# Autodesk Inventor assembly: 1_Base
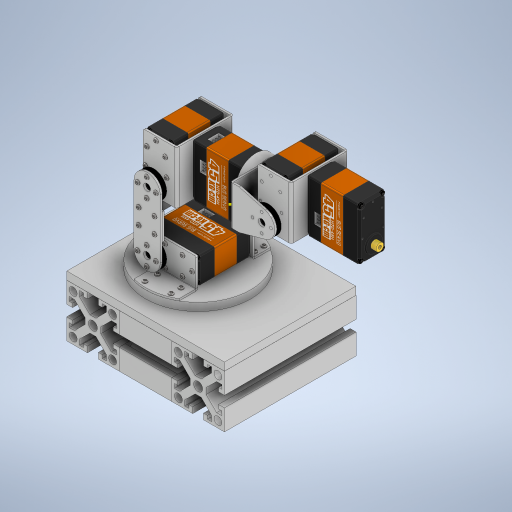
[picture p0: Inventor's stored thumbnail of the model, 512x512]
Saved by Autodesk Inventor 2024.1 (Build 281209000, 209)
## iProperties
Created: 2023-08-24
Part Number: 1_Base
Document SubType Name: Assembly
Designer: chanh
Author: chanh
## Documents named in this file (28)
- C:\Users\chanh\OneDrive - 연세대학교 (Yonsei University)\로봇\Humanoid\Roboin Humanoid Project\Inventor\rh_plus_7_axis_robot_arm_hardware\Assembly\2_Arm.iam
- C:\Users\chanh\OneDrive - 연세대학교 (Yonsei University)\로봇\Humanoid\Roboin Humanoid Project\Inventor\rh_plus_7_axis_robot_arm_hardware\Part\HTD-45H, Horn\HTD-45H\HTD-45H.ipt
- C:\Users\chanh\OneDrive - 연세대학교 (Yonsei University)\로봇\Humanoid\Roboin Humanoid Project\Inventor\rh_plus_7_axis_robot_arm_hardware\Part\Frame\axis_1_top_frame.ipt
- C:\Users\chanh\OneDrive - 연세대학교 (Yonsei University)\로봇\Humanoid\Roboin Humanoid Project\Inventor\rh_plus_7_axis_robot_arm_hardware\Part\Other Parts\Aluminum_Profile_4040_100.14mm_top.ipt
- C:\Users\chanh\OneDrive - 연세대학교 (Yonsei University)\로봇\Humanoid\Roboin Humanoid Project\Inventor\rh_plus_7_axis_robot_arm_hardware\Part\Other Parts\Aluminum_Profile_4040_40.10mm_right.ipt
- C:\Users\chanh\OneDrive - 연세대학교 (Yonsei University)\로봇\Humanoid\Roboin Humanoid Project\Inventor\rh_plus_7_axis_robot_arm_hardware\Part\Other Parts\Aluminum_Profile_4040_40.10mm_left.ipt
- C:\Users\chanh\OneDrive - 연세대학교 (Yonsei University)\로봇\Humanoid\Roboin Humanoid Project\Inventor\rh_plus_7_axis_robot_arm_hardware\Part\Other Parts\Aluminum_Profile_4040_100.14mm_bottom.ipt
- C:\Users\chanh\OneDrive - 연세대학교 (Yonsei University)\로봇\Humanoid\Roboin Humanoid Project\Inventor\rh_plus_7_axis_robot_arm_hardware\Part\HTD-45H, Horn\HTD-45H\M2x32.ipt
- C:\Users\chanh\OneDrive - 연세대학교 (Yonsei University)\로봇\Humanoid\Roboin Humanoid Project\Inventor\rh_plus_7_axis_robot_arm_hardware\Part\HTD-45H, Horn\Horn\Top Horn.ipt
- C:\Users\chanh\OneDrive - 연세대학교 (Yonsei University)\로봇\Humanoid\Roboin Humanoid Project\Inventor\rh_plus_7_axis_robot_arm_hardware\Part\Bolt, Bearing\M2x6 Round Bolt.ipt
- C:\Users\chanh\OneDrive - 연세대학교 (Yonsei University)\로봇\Humanoid\Roboin Humanoid Project\Inventor\rh_plus_7_axis_robot_arm_hardware\Part\Bolt, Bearing\M2x35 Round Bolt.ipt
- C:\Users\chanh\OneDrive - 연세대학교 (Yonsei University)\로봇\Humanoid\Roboin Humanoid Project\Inventor\rh_plus_7_axis_robot_arm_hardware\Part\Frame\axis_2_bottom_frame.ipt
- C:\Users\chanh\OneDrive - 연세대학교 (Yonsei University)\로봇\Humanoid\Roboin Humanoid Project\Inventor\rh_plus_7_axis_robot_arm_hardware\Part\Bolt, Bearing\AXK5070+AS Bearing.ipt
- C:\Users\chanh\OneDrive - 연세대학교 (Yonsei University)\로봇\Humanoid\Roboin Humanoid Project\Inventor\rh_plus_7_axis_robot_arm_hardware\Part\Bolt, Bearing\M2x6 Bolt.ipt
- C:\Users\chanh\OneDrive - 연세대학교 (Yonsei University)\로봇\Humanoid\Roboin Humanoid Project\Inventor\rh_plus_7_axis_robot_arm_hardware\Part\HTD-45H, Horn\HTD-45H\HTD-45H.iam
- C:\Users\chanh\OneDrive - 연세대학교 (Yonsei University)\로봇\Humanoid\Roboin Humanoid Project\Inventor\rh_plus_7_axis_robot_arm_hardware\Part\HTD-45H, Horn\Horn\M3x6.ipt
- C:\Users\chanh\OneDrive - 연세대학교 (Yonsei University)\로봇\Humanoid\Roboin Humanoid Project\Inventor\rh_plus_7_axis_robot_arm_hardware\Part\Frame\axis_2_bottom_L_frame(top).ipt
- C:\Users\chanh\OneDrive - 연세대학교 (Yonsei University)\로봇\Humanoid\Roboin Humanoid Project\Inventor\rh_plus_7_axis_robot_arm_hardware\Part\Frame\axis_2_bottom_L_frame(bottom).ipt
- C:\Users\chanh\OneDrive - 연세대학교 (Yonsei University)\로봇\Humanoid\Roboin Humanoid Project\Inventor\rh_plus_7_axis_robot_arm_hardware\Part\HTD-45H, Horn\Horn\Bottom Horn.ipt
- C:\Users\chanh\OneDrive - 연세대학교 (Yonsei University)\로봇\Humanoid\Roboin Humanoid Project\Inventor\rh_plus_7_axis_robot_arm_hardware\Part\Bolt, Bearing\M2x4 Round Bolt.ipt
- C:\Users\chanh\OneDrive - 연세대학교 (Yonsei University)\로봇\Humanoid\Roboin Humanoid Project\Inventor\rh_plus_7_axis_robot_arm_hardware\Part\Frame\axis_3_bottom_frame(top).ipt
- C:\Users\chanh\OneDrive - 연세대학교 (Yonsei University)\로봇\Humanoid\Roboin Humanoid Project\Inventor\rh_plus_7_axis_robot_arm_hardware\Part\Frame\axis_3_bottom_frame(bottom).ipt
- C:\Users\chanh\OneDrive - 연세대학교 (Yonsei University)\로봇\Humanoid\Roboin Humanoid Project\Inventor\rh_plus_7_axis_robot_arm_hardware\Part\Frame\axis_3_bottom_frame(middle).ipt
- C:\Users\chanh\OneDrive - 연세대학교 (Yonsei University)\로봇\Humanoid\Roboin Humanoid Project\Inventor\rh_plus_7_axis_robot_arm_hardware\Part\Frame\axis_3_top_frame.ipt
- C:\Users\chanh\OneDrive - 연세대학교 (Yonsei University)\로봇\Humanoid\Roboin Humanoid Project\Inventor\rh_plus_7_axis_robot_arm_hardware\Part\Frame\axis_4_top_frame.ipt
- C:\Users\chanh\OneDrive - 연세대학교 (Yonsei University)\로봇\Humanoid\Roboin Humanoid Project\Inventor\rh_plus_7_axis_robot_arm_hardware\Part\Bolt, Bearing\2030 Teflon Sheet.ipt
- C:\Users\chanh\OneDrive - 연세대학교 (Yonsei University)\로봇\Humanoid\Roboin Humanoid Project\Inventor\rh_plus_7_axis_robot_arm_hardware\Part\Frame\axis_5_bottom_frame.ipt
- C:\Users\chanh\OneDrive - 연세대학교 (Yonsei University)\로봇\Humanoid\Roboin Humanoid Project\Inventor\rh_plus_7_axis_robot_arm_hardware\Part\Frame\axis_5_top_frame.ipt
## Components (113 placed, 26 different names)
1. Aluminum_Profile_4040_100.14mm_top:1 — Flush:13, Flush:14, Mate:2, Mate:3, Flush:15, Flush:16, Mate:4, Flush:17, Flush:18, Mate:6
2. Aluminum_Profile_4040_40.10mm_right:1 — Mate:3, Flush:15, Flush:16
3. Aluminum_Profile_4040_40.10mm_left:1 — Mate:4, Flush:17, Flush:18, Mate:5, Flush:20
4. Aluminum_Profile_4040_100.14mm_bottom:1 — Flush:19, Mate:5, Flush:20
5. HTD-45H:1 — Mate:1, Flush:1, Flush:2, Flush:12, Flush:13, Flush:14, Mate:2, Flush:19, Rigid:1, Rigid:2, Rotational:1, Mate:7, Mate:8
6. axis_1_top_frame:1 — Flush:11, Flush:12, Mate:6, Rigid:11, Rigid:12, Rigid:13, Rigid:14, Rigid:15, Rigid:16, Rigid:17, Mate:9
7. HTD-45H:2 [sub-assembly] — Flush:21, Mate:11, Flush:23, Flush:24, Mate:13, Mate:17, Rotational:2
8. axis_2_bottom_frame:1 — Rigid:10, Rigid:18, Rigid:19, Rigid:20, Rigid:21, Flush:21, Mate:11, Mate:14
9. axis_2_bottom_L_frame(top):1 — Flush:23, Flush:24, Mate:13, Mate:14, Rigid:23, Rigid:24, Rigid:25, Rigid:26, Rigid:27, Rigid:28, Rigid:29, Rigid:30, Rigid:31
10. axis_2_bottom_L_frame(bottom):1 — Mate:17, Rigid:32, Rigid:33, Rigid:34, Rigid:35, Rigid:36, Rigid:37, Rigid:38, Rigid:39, Rigid:40, Rigid:41, Rigid:42, Rigid:43
11. HTD-45H:3 [sub-assembly] — Rotational:3, Flush:25, Mate:18, Flush:26
12. axis_3_bottom_frame(top):1 — Rigid:44, Rigid:45, Rigid:48, Rigid:49, Rigid:50, Rigid:51, Rigid:52, Rigid:53, Rigid:54, Rigid:55, Rigid:56, Rigid:57, Rigid:58, Rigid:59, Rigid:60
13. axis_3_bottom_frame(middle):1 — Rigid:48, Rigid:104
14. axis_3_bottom_frame(bottom):1 — Rigid:61, Rigid:62, Rigid:63, Rigid:64, Rigid:65, Rigid:66, Rigid:67, Rigid:68, Rigid:69, Rigid:70, Rigid:71, Rigid:72, Rigid:102, Rigid:103, Rigid:104
15. axis_3_top_frame:1 — Flush:25, Mate:18, Flush:26, Rigid:74, Rigid:75, Rigid:76, Rigid:77, Rigid:78, Rigid:79, Rigid:80, Rigid:81, Rigid:82, Rigid:83, Rigid:84, Rigid:85, Rigid:86, Rigid:87, Rigid:88, Rigid:89, Rigid:90
16. HTD-45H:4 — Rigid:90, Rigid:91, Rigid:92, Angle:1, Mate:20, Rotational:4
17. 2030 Teflon Sheet:1 — Rigid:97
18. axis_4_top_frame:1 — Angle:1, Mate:20, Rigid:93, Rigid:94, Rigid:95, Rigid:96, Rigid:97
19. HTD-45H:5 [sub-assembly] — Rotational:5, Rigid:105
20. 2030 Teflon Sheet:2
21. axis_5_bottom_frame:1 — Rigid:99, Rigid:100, Rigid:101
22. axis_5_top_frame:1 — Rigid:105, Mate:21, Flush:27, Mate:22
23. HTD-45H:6 [sub-assembly] — Mate:21, Flush:27, Mate:22
24. M2x32:1 — Rigid:2
25. M2x32:2 — Rigid:1
26. Top Horn:1 — Rotational:1, Rigid:10, Rigid:22
27. M3x6:1 — Rigid:22
28. M2x6 Round Bolt:3 — Rigid:16
29. M2x6 Round Bolt:4 — Rigid:17
30. M2x6 Round Bolt:5 — Rigid:15
31. AXK5070+AS Bearing:1 — Mate:7, Mate:8, Mate:9
32. M2x6 Round Bolt:1 — Rigid:14
33. M2x6 Round Bolt:2 — Rigid:13
34. M2x35 Round Bolt:1 — Rigid:11
35. M2x35 Round Bolt:2 — Rigid:12
36. Bottom Horn:5 — Rigid:102
37. Top Horn:2 — Rotational:2, Rigid:44
38. M2x6 Bolt:1 — Rigid:18
39. M2x6 Bolt:2 — Rigid:19
40. M2x6 Bolt:3 — Rigid:20
41. M2x6 Bolt:4 — Rigid:21
42. M2x4 Round Bolt:1 — Rigid:23
43. M2x4 Round Bolt:2 — Rigid:24
44. M2x4 Round Bolt:3 — Rigid:25
45. M2x4 Round Bolt:4 — Rigid:26
46. M2x4 Round Bolt:5 — Rigid:27
47. M2x4 Round Bolt:6 — Rigid:28
48. M2x4 Round Bolt:7 — Rigid:29
49. M2x4 Round Bolt:8 — Rigid:30
50. M2x4 Round Bolt:9 — Rigid:31
51. M2x4 Round Bolt:10 — Rigid:32
52. M2x4 Round Bolt:11 — Rigid:33
53. M2x4 Round Bolt:12 — Rigid:34
54. M2x4 Round Bolt:13 — Rigid:35
55. M2x4 Round Bolt:14 — Rigid:36
56. M2x4 Round Bolt:15 — Rigid:37
57. M2x4 Round Bolt:16 — Rigid:38
58. M2x4 Round Bolt:17 — Rigid:39
59. M2x4 Round Bolt:18 — Rigid:40
60. M2x4 Round Bolt:19 — Rigid:41
61. M2x4 Round Bolt:20 — Rigid:42
62. M2x4 Round Bolt:21 — Rigid:43
63. Bottom Horn:4 — Rigid:103
64. Top Horn:3 — Rotational:3, Rigid:45
65. M2x4 Round Bolt:22 — Rigid:50
66. M2x4 Round Bolt:23 — Rigid:51
67. M2x4 Round Bolt:24 — Rigid:52
68. M2x4 Round Bolt:25 — Rigid:49
69. M2x4 Round Bolt:26 — Rigid:53
70. M2x4 Round Bolt:27 — Rigid:54
71. M2x4 Round Bolt:28 — Rigid:55
72. M2x4 Round Bolt:29 — Rigid:56
73. M2x4 Round Bolt:30 — Rigid:57
74. M2x4 Round Bolt:31 — Rigid:58
75. M2x4 Round Bolt:32 — Rigid:59
76. M2x4 Round Bolt:33 — Rigid:60
77. M2x4 Round Bolt:34 — Rigid:61
78. M2x4 Round Bolt:35 — Rigid:62
79. M2x4 Round Bolt:36 — Rigid:63
80. M2x4 Round Bolt:37 — Rigid:64
81. M2x4 Round Bolt:38 — Rigid:65
82. M2x4 Round Bolt:39 — Rigid:66
83. M2x4 Round Bolt:40 — Rigid:67
84. M2x4 Round Bolt:41 — Rigid:68
85. M2x4 Round Bolt:42 — Rigid:69
86. M2x4 Round Bolt:43 — Rigid:70
87. M2x4 Round Bolt:44 — Rigid:71
88. M2x4 Round Bolt:45 — Rigid:72
89. M2x4 Round Bolt:46 — Rigid:74
90. M2x4 Round Bolt:47 — Rigid:75
91. M2x4 Round Bolt:48 — Rigid:76
92. M2x4 Round Bolt:49 — Rigid:77
93. M2x4 Round Bolt:50 — Rigid:78
94. M2x4 Round Bolt:51 — Rigid:79
95. M2x4 Round Bolt:52 — Rigid:80
96. M2x4 Round Bolt:53 — Rigid:81
97. M2x4 Round Bolt:54 — Rigid:82
98. M2x4 Round Bolt:55 — Rigid:83
99. M2x4 Round Bolt:56 — Rigid:84
100. M2x4 Round Bolt:57 — Rigid:85
101. M2x4 Round Bolt:58 — Rigid:86
102. M2x4 Round Bolt:59 — Rigid:87
103. M2x4 Round Bolt:60 — Rigid:88
104. M2x4 Round Bolt:61 — Rigid:89
105. Top Horn:6 — Rotational:4, Rigid:99
106. M2x32:3 — Rigid:92
107. M2x32:4 — Rigid:91
108. M2x6 Round Bolt:6 — Rigid:93
109. M2x6 Round Bolt:7 — Rigid:94
110. M2x35 Round Bolt:3 — Rigid:95
111. M2x35 Round Bolt:4 — Rigid:96
112. Top Horn:7 — Rigid:100, Rotational:5
113. Bottom Horn:3 — Rigid:101
## Relationships (135: WeldJoint 94, Flush 18, Mate 17, RevoluteJoint 5, Angle 1)
- Mate:1: HTD-45H:1
- Flush:1: HTD-45H:1
- Flush:2: HTD-45H:1
- Flush:11: axis_1_top_frame:1
- Flush:12: HTD-45H:1 ↔ axis_1_top_frame:1
- Flush:13: Aluminum_Profile_4040_100.14mm_top:1 ↔ HTD-45H:1
- Flush:14: Aluminum_Profile_4040_100.14mm_top:1 ↔ HTD-45H:1
- Mate:2: Aluminum_Profile_4040_100.14mm_top:1 ↔ HTD-45H:1
- Mate:3: Aluminum_Profile_4040_100.14mm_top:1 ↔ Aluminum_Profile_4040_40.10mm_right:1
- Flush:15: Aluminum_Profile_4040_100.14mm_top:1 ↔ Aluminum_Profile_4040_40.10mm_right:1
- Flush:16: Aluminum_Profile_4040_100.14mm_top:1 ↔ Aluminum_Profile_4040_40.10mm_right:1
- Mate:4: Aluminum_Profile_4040_100.14mm_top:1 ↔ Aluminum_Profile_4040_40.10mm_left:1
- Flush:17: Aluminum_Profile_4040_100.14mm_top:1 ↔ Aluminum_Profile_4040_40.10mm_left:1
- Flush:18: Aluminum_Profile_4040_100.14mm_top:1 ↔ Aluminum_Profile_4040_40.10mm_left:1
- Flush:19: Aluminum_Profile_4040_100.14mm_bottom:1 ↔ HTD-45H:1
- Mate:5: Aluminum_Profile_4040_40.10mm_left:1 ↔ Aluminum_Profile_4040_100.14mm_bottom:1
- Flush:20: Aluminum_Profile_4040_40.10mm_left:1 ↔ Aluminum_Profile_4040_100.14mm_bottom:1
- Mate:6: Aluminum_Profile_4040_100.14mm_top:1 ↔ axis_1_top_frame:1
- Rigid:1 [WeldJoint]: HTD-45H:1 ↔ M2x32:2
- Rigid:2 [WeldJoint]: HTD-45H:1 ↔ M2x32:1
- Rotational:1 [RevoluteJoint]: HTD-45H:1 ↔ Top Horn:1
- Rigid:10 [WeldJoint]: axis_2_bottom_frame:1 ↔ Top Horn:1
- Rigid:11 [WeldJoint]: axis_1_top_frame:1 ↔ M2x35 Round Bolt:1
- Rigid:12 [WeldJoint]: axis_1_top_frame:1 ↔ M2x35 Round Bolt:2
- Rigid:13 [WeldJoint]: axis_1_top_frame:1 ↔ M2x6 Round Bolt:2
- Rigid:14 [WeldJoint]: axis_1_top_frame:1 ↔ M2x6 Round Bolt:1
- Rigid:15 [WeldJoint]: axis_1_top_frame:1 ↔ M2x6 Round Bolt:5
- Rigid:16 [WeldJoint]: axis_1_top_frame:1 ↔ M2x6 Round Bolt:3
- Rigid:17 [WeldJoint]: axis_1_top_frame:1 ↔ M2x6 Round Bolt:4
- Mate:7: HTD-45H:1 ↔ AXK5070+AS Bearing:1
- Mate:8: HTD-45H:1 ↔ AXK5070+AS Bearing:1
- Mate:9: axis_1_top_frame:1 ↔ AXK5070+AS Bearing:1
- Rigid:18 [WeldJoint]: axis_2_bottom_frame:1 ↔ M2x6 Bolt:1
- Rigid:19 [WeldJoint]: axis_2_bottom_frame:1 ↔ M2x6 Bolt:2
- Rigid:20 [WeldJoint]: axis_2_bottom_frame:1 ↔ M2x6 Bolt:3
- Rigid:21 [WeldJoint]: axis_2_bottom_frame:1 ↔ M2x6 Bolt:4
- Rigid:22 [WeldJoint]: Top Horn:1 ↔ M3x6:1
- Flush:21: HTD-45H:2 ↔ axis_2_bottom_frame:1
- Mate:11: HTD-45H:2 ↔ axis_2_bottom_frame:1
- Flush:23: HTD-45H:2 ↔ axis_2_bottom_L_frame(top):1
- Flush:24 (-1 mm): HTD-45H:2 ↔ axis_2_bottom_L_frame(top):1
- Mate:13: HTD-45H:2 ↔ axis_2_bottom_L_frame(top):1
- Mate:14: axis_2_bottom_frame:1 ↔ axis_2_bottom_L_frame(top):1
- Mate:17: HTD-45H:2 ↔ axis_2_bottom_L_frame(bottom):1
- Rotational:2 [RevoluteJoint]: HTD-45H:2 ↔ Top Horn:2
- Rigid:23 [WeldJoint]: axis_2_bottom_L_frame(top):1 ↔ M2x4 Round Bolt:1
- Rigid:24 [WeldJoint]: axis_2_bottom_L_frame(top):1 ↔ M2x4 Round Bolt:2
- Rigid:25 [WeldJoint]: axis_2_bottom_L_frame(top):1 ↔ M2x4 Round Bolt:3
- Rigid:26 [WeldJoint]: axis_2_bottom_L_frame(top):1 ↔ M2x4 Round Bolt:4
- Rigid:27 [WeldJoint]: axis_2_bottom_L_frame(top):1 ↔ M2x4 Round Bolt:5
- Rigid:28 [WeldJoint]: axis_2_bottom_L_frame(top):1 ↔ M2x4 Round Bolt:6
- Rigid:29 [WeldJoint]: axis_2_bottom_L_frame(top):1 ↔ M2x4 Round Bolt:7
- Rigid:30 [WeldJoint]: axis_2_bottom_L_frame(top):1 ↔ M2x4 Round Bolt:8
- Rigid:31 [WeldJoint]: axis_2_bottom_L_frame(top):1 ↔ M2x4 Round Bolt:9
- Rigid:32 [WeldJoint]: axis_2_bottom_L_frame(bottom):1 ↔ M2x4 Round Bolt:10
- Rigid:33 [WeldJoint]: axis_2_bottom_L_frame(bottom):1 ↔ M2x4 Round Bolt:11
- Rigid:34 [WeldJoint]: axis_2_bottom_L_frame(bottom):1 ↔ M2x4 Round Bolt:12
- Rigid:35 [WeldJoint]: axis_2_bottom_L_frame(bottom):1 ↔ M2x4 Round Bolt:13
- Rigid:36 [WeldJoint]: axis_2_bottom_L_frame(bottom):1 ↔ M2x4 Round Bolt:14
- Rigid:37 [WeldJoint]: axis_2_bottom_L_frame(bottom):1 ↔ M2x4 Round Bolt:15
- Rigid:38 [WeldJoint]: axis_2_bottom_L_frame(bottom):1 ↔ M2x4 Round Bolt:16
- Rigid:39 [WeldJoint]: axis_2_bottom_L_frame(bottom):1 ↔ M2x4 Round Bolt:17
- Rigid:40 [WeldJoint]: axis_2_bottom_L_frame(bottom):1 ↔ M2x4 Round Bolt:18
- Rigid:41 [WeldJoint]: axis_2_bottom_L_frame(bottom):1 ↔ M2x4 Round Bolt:19
- Rigid:42 [WeldJoint]: axis_2_bottom_L_frame(bottom):1 ↔ M2x4 Round Bolt:20
- Rigid:43 [WeldJoint]: axis_2_bottom_L_frame(bottom):1 ↔ M2x4 Round Bolt:21
- Rotational:3 [RevoluteJoint]: HTD-45H:3 ↔ Top Horn:3
- Rigid:44 [WeldJoint]: axis_3_bottom_frame(top):1 ↔ Top Horn:2
- Rigid:45 [WeldJoint]: axis_3_bottom_frame(top):1 ↔ Top Horn:3
- Rigid:48 [WeldJoint]: axis_3_bottom_frame(top):1 ↔ axis_3_bottom_frame(middle):1
- Rigid:49 [WeldJoint]: axis_3_bottom_frame(top):1 ↔ M2x4 Round Bolt:25
- Rigid:50 [WeldJoint]: axis_3_bottom_frame(top):1 ↔ M2x4 Round Bolt:22
- Rigid:51 [WeldJoint]: axis_3_bottom_frame(top):1 ↔ M2x4 Round Bolt:23
- Rigid:52 [WeldJoint]: axis_3_bottom_frame(top):1 ↔ M2x4 Round Bolt:24
- Rigid:53 [WeldJoint]: axis_3_bottom_frame(top):1 ↔ M2x4 Round Bolt:26
- Rigid:54 [WeldJoint]: axis_3_bottom_frame(top):1 ↔ M2x4 Round Bolt:27
- Rigid:55 [WeldJoint]: axis_3_bottom_frame(top):1 ↔ M2x4 Round Bolt:28
- Rigid:56 [WeldJoint]: axis_3_bottom_frame(top):1 ↔ M2x4 Round Bolt:29
- Rigid:57 [WeldJoint]: axis_3_bottom_frame(top):1 ↔ M2x4 Round Bolt:30
- Rigid:58 [WeldJoint]: axis_3_bottom_frame(top):1 ↔ M2x4 Round Bolt:31
- Rigid:59 [WeldJoint]: axis_3_bottom_frame(top):1 ↔ M2x4 Round Bolt:32
- Rigid:60 [WeldJoint]: axis_3_bottom_frame(top):1 ↔ M2x4 Round Bolt:33
- Rigid:61 [WeldJoint]: axis_3_bottom_frame(bottom):1 ↔ M2x4 Round Bolt:34
- Rigid:62 [WeldJoint]: axis_3_bottom_frame(bottom):1 ↔ M2x4 Round Bolt:35
- Rigid:63 [WeldJoint]: axis_3_bottom_frame(bottom):1 ↔ M2x4 Round Bolt:36
- Rigid:64 [WeldJoint]: axis_3_bottom_frame(bottom):1 ↔ M2x4 Round Bolt:37
- Rigid:65 [WeldJoint]: axis_3_bottom_frame(bottom):1 ↔ M2x4 Round Bolt:38
- Rigid:66 [WeldJoint]: axis_3_bottom_frame(bottom):1 ↔ M2x4 Round Bolt:39
- Rigid:67 [WeldJoint]: axis_3_bottom_frame(bottom):1 ↔ M2x4 Round Bolt:40
- Rigid:68 [WeldJoint]: axis_3_bottom_frame(bottom):1 ↔ M2x4 Round Bolt:41
- Rigid:69 [WeldJoint]: axis_3_bottom_frame(bottom):1 ↔ M2x4 Round Bolt:42
- Rigid:70 [WeldJoint]: axis_3_bottom_frame(bottom):1 ↔ M2x4 Round Bolt:43
- Rigid:71 [WeldJoint]: axis_3_bottom_frame(bottom):1 ↔ M2x4 Round Bolt:44
- Rigid:72 [WeldJoint]: axis_3_bottom_frame(bottom):1 ↔ M2x4 Round Bolt:45
- Flush:25: HTD-45H:3 ↔ axis_3_top_frame:1
- Mate:18: HTD-45H:3 ↔ axis_3_top_frame:1
- Flush:26: HTD-45H:3 ↔ axis_3_top_frame:1
- Rigid:74 [WeldJoint]: axis_3_top_frame:1 ↔ M2x4 Round Bolt:46
- Rigid:75 [WeldJoint]: axis_3_top_frame:1 ↔ M2x4 Round Bolt:47
- Rigid:76 [WeldJoint]: axis_3_top_frame:1 ↔ M2x4 Round Bolt:48
- Rigid:77 [WeldJoint]: axis_3_top_frame:1 ↔ M2x4 Round Bolt:49
- Rigid:78 [WeldJoint]: axis_3_top_frame:1 ↔ M2x4 Round Bolt:50
- Rigid:79 [WeldJoint]: axis_3_top_frame:1 ↔ M2x4 Round Bolt:51
- Rigid:80 [WeldJoint]: axis_3_top_frame:1 ↔ M2x4 Round Bolt:52
- Rigid:81 [WeldJoint]: axis_3_top_frame:1 ↔ M2x4 Round Bolt:53
- Rigid:82 [WeldJoint]: axis_3_top_frame:1 ↔ M2x4 Round Bolt:54
- Rigid:83 [WeldJoint]: axis_3_top_frame:1 ↔ M2x4 Round Bolt:55
- Rigid:84 [WeldJoint]: axis_3_top_frame:1 ↔ M2x4 Round Bolt:56
- Rigid:85 [WeldJoint]: axis_3_top_frame:1 ↔ M2x4 Round Bolt:57
- Rigid:86 [WeldJoint]: axis_3_top_frame:1 ↔ M2x4 Round Bolt:58
- Rigid:87 [WeldJoint]: axis_3_top_frame:1 ↔ M2x4 Round Bolt:59
- Rigid:88 [WeldJoint]: axis_3_top_frame:1 ↔ M2x4 Round Bolt:60
- Rigid:89 [WeldJoint]: axis_3_top_frame:1 ↔ M2x4 Round Bolt:61
- Rigid:90 [WeldJoint]: axis_3_top_frame:1 ↔ HTD-45H:4
- Rigid:91 [WeldJoint]: HTD-45H:4 ↔ M2x32:4
- Rigid:92 [WeldJoint]: HTD-45H:4 ↔ M2x32:3
- Angle:1 (0 deg): HTD-45H:4 ↔ axis_4_top_frame:1
- Mate:20: HTD-45H:4 ↔ axis_4_top_frame:1
- Rigid:93 [WeldJoint]: axis_4_top_frame:1 ↔ M2x6 Round Bolt:6
- Rigid:94 [WeldJoint]: axis_4_top_frame:1 ↔ M2x6 Round Bolt:7
- Rigid:95 [WeldJoint]: axis_4_top_frame:1 ↔ M2x35 Round Bolt:3
- Rigid:96 [WeldJoint]: axis_4_top_frame:1 ↔ M2x35 Round Bolt:4
- Rigid:97 [WeldJoint]: 2030 Teflon Sheet:1 ↔ axis_4_top_frame:1
- Rotational:4 [RevoluteJoint]: HTD-45H:4 ↔ Top Horn:6
- Rigid:99 [WeldJoint]: axis_5_bottom_frame:1 ↔ Top Horn:6
- Rigid:100 [WeldJoint]: axis_5_bottom_frame:1 ↔ Top Horn:7
- Rigid:101 [WeldJoint]: axis_5_bottom_frame:1 ↔ Bottom Horn:3
- Rotational:5 [RevoluteJoint]: HTD-45H:5 ↔ Top Horn:7
- Rigid:102 [WeldJoint]: axis_3_bottom_frame(bottom):1 ↔ Bottom Horn:5
- Rigid:103 [WeldJoint]: axis_3_bottom_frame(bottom):1 ↔ Bottom Horn:4
- Rigid:104 [WeldJoint]: axis_3_bottom_frame(middle):1 ↔ axis_3_bottom_frame(bottom):1
- Rigid:105 [WeldJoint]: HTD-45H:5 ↔ axis_5_top_frame:1
- Mate:21: axis_5_top_frame:1 ↔ HTD-45H:6
- Flush:27: axis_5_top_frame:1 ↔ HTD-45H:6
- Mate:22: axis_5_top_frame:1 ↔ HTD-45H:6
